# Autodesk Inventor assembly: これで完成パネル型スカラアーム
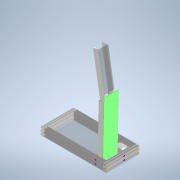
[picture p0: Inventor's stored thumbnail of the model, 180x180]
Saved by Autodesk Inventor 2022 (Build 260153000, 153)
## iProperties
Created: 2022-12-16
Part Number: これで完成パネル型スカラアーム
Document SubType Name: Assembly
Designer: tdn82
Author: tdn82
## Documents named in this file (21)
- C:\Users\tdn82\OneDrive\ドキュメント\Inventor\卒業研究パネル型スカラアーム\GrabCAD\panel-type-scalar-arm\パネル型スカラアーム\サーボ固定パーツ３Dプリンタ出力実験\これで完成パネル型スカラアーム.iam
- C:\Users\tdn82\OneDrive\ドキュメント\Inventor\卒業研究パネル型スカラアーム\GrabCAD\panel-type-scalar-arm\パネル型スカラアーム\後ろカバー.ipt
- C:\Users\tdn82\OneDrive\ドキュメント\Inventor\卒業研究パネル型スカラアーム\GrabCAD\panel-type-scalar-arm\パネル型スカラアーム\HFS5-2040-180-Z5-YA10-YB99-YC170.ipt
- C:\Users\tdn82\OneDrive\ドキュメント\Inventor\卒業研究パネル型スカラアーム\GrabCAD\panel-type-scalar-arm\パネル型スカラアーム\HFS5-2040-320-TPW-Z5-YA42_5.ipt
- C:\Users\tdn82\OneDrive\ドキュメント\Inventor\卒業研究パネル型スカラアーム\GrabCAD\panel-type-scalar-arm\パネル型スカラアーム\HFS5-2040-320-TPW.ipt
- C:\Users\tdn82\OneDrive\ドキュメント\Inventor\卒業研究パネル型スカラアーム\GrabCAD\panel-type-scalar-arm\パネル型スカラアーム\HFS5-2040-180-Z5-YA10-YB170-Left.ipt
- C:\Users\tdn82\OneDrive\ドキュメント\Inventor\卒業研究パネル型スカラアーム\GrabCAD\panel-type-scalar-arm\パネル型スカラアーム\サーボ固定パーツ３Dプリンタ出力実験\サーボモータ固定用１軸目.ipt
- C:\Users\tdn82\OneDrive\ドキュメント\Inventor\卒業研究パネル型スカラアーム\GrabCAD\panel-type-scalar-arm\パネル型スカラアーム\サーボモータB3M1000_scale.ipt
- C:\Users\tdn82\OneDrive\ドキュメント\Inventor\卒業研究パネル型スカラアーム\GrabCAD\panel-type-scalar-arm\パネル型スカラアーム\サーボ固定パーツ３Dプリンタ出力実験\シャフト固定用.ipt
- C:\Users\tdn82\OneDrive\ドキュメント\Inventor\卒業研究パネル型スカラアーム\GrabCAD\panel-type-scalar-arm\パネル型スカラアーム\横長2ndフラットバー上 アルミフレーム用.ipt
- C:\Users\tdn82\OneDrive\ドキュメント\Inventor\卒業研究パネル型スカラアーム\GrabCAD\panel-type-scalar-arm\パネル型スカラアーム\横長2ndフラットバー下 アルミフレーム用.ipt
- C:\Users\tdn82\OneDrive\ドキュメント\Inventor\卒業研究パネル型スカラアーム\GrabCAD\panel-type-scalar-arm\パネル型スカラアーム\前カバー中盤左アーム固定.ipt
- C:\Users\tdn82\OneDrive\ドキュメント\Inventor\卒業研究パネル型スカラアーム\GrabCAD\panel-type-scalar-arm\パネル型スカラアーム\サーボ固定パーツ３Dプリンタ出力実験\サーボモータ固定用２軸目3mm改_new.ipt
- C:\Users\tdn82\OneDrive\ドキュメント\Inventor\卒業研究パネル型スカラアーム\GrabCAD\panel-type-scalar-arm\パネル型スカラアーム\アルミフリーホーン02137_AluminumFreeHornWithBearing_B3M_6000.ipt
- C:\Users\tdn82\OneDrive\ドキュメント\Inventor\卒業研究パネル型スカラアーム\GrabCAD\panel-type-scalar-arm\パネル型スカラアーム\シャフト.ipt
- C:\Users\tdn82\OneDrive\ドキュメント\Inventor\卒業研究パネル型スカラアーム\GrabCAD\panel-type-scalar-arm\パネル型スカラアーム\FL674ZZ.ipt
- C:\Users\tdn82\OneDrive\ドキュメント\Inventor\卒業研究パネル型スカラアーム\GrabCAD\panel-type-scalar-arm\パネル型スカラアーム\シャフトカラー.ipt
- C:\Users\tdn82\OneDrive\ドキュメント\Inventor\卒業研究パネル型スカラアーム\GrabCAD\panel-type-scalar-arm\パネル型スカラアーム\横長3rdフラットバー下.ipt
- C:\Users\tdn82\OneDrive\ドキュメント\Inventor\卒業研究パネル型スカラアーム\GrabCAD\panel-type-scalar-arm\パネル型スカラアーム\三段目アクリル板.ipt
- C:\Users\tdn82\OneDrive\ドキュメント\Inventor\卒業研究パネル型スカラアーム\GrabCAD\panel-type-scalar-arm\パネル型スカラアーム\CBE5-25.ipt
- C:\Users\tdn82\OneDrive\ドキュメント\Inventor\卒業研究パネル型スカラアーム\GrabCAD\panel-type-scalar-arm\パネル型スカラアーム\CBE5-20.ipt
## Components (32 placed, 20 different names)
1. 後ろカバー:3 — メイト:1, メイト:2, フラッシュ:1, メイト:3, フラッシュ:2, フラッシュ:4, メイト:17
2. HFS5-2040-180-Z5-YA10-YB99-YC170:1 — メイト:3, フラッシュ:2, メイト:6, フラッシュ:4, メイト:9, フラッシュ:6, メイト:11, 挿入:26, 挿入:27, 挿入:28, 挿入:29, 挿入:30, 挿入:31, フラッシュ:9, メイト:18, フラッシュ:10
3. HFS5-2040-320-TPW-Z5-YA42_5:1 — フラッシュ:9, メイト:18, フラッシュ:10, 挿入:32, 挿入:33, メイト:19, メイト:22
4. HFS5-2040-320-TPW:1 — メイト:2, フラッシュ:1, メイト:6, メイト:16, フラッシュ:8
5. HFS5-2040-180-Z5-YA10-YB170-Left:1 — メイト:16, メイト:17, フラッシュ:8, 挿入:22, 挿入:23, 挿入:24, 挿入:25
6. サーボモータ固定用１軸目:1 — メイト:9, フラッシュ:6, メイト:10, 挿入:1, 挿入:2, メイト:11
7. サーボモータB3M1000_scale:1 — メイト:10, 挿入:1, 挿入:2, 挿入:12
8. サーボモータB3M1000_scale:2 — 挿入:9, 挿入:10, 挿入:18, 挿入:19, 挿入:20
9. シャフト固定用:1 — メイト:19, メイト:20, メイト:21
10. 横長2ndフラットバー上 アルミフレーム用:1 — 挿入:3, 挿入:4, 挿入:12
11. 横長2ndフラットバー下 アルミフレーム用:1 — 挿入:13, 挿入:14, 挿入:15
12. 前カバー中盤左アーム固定:1 — 挿入:3, 挿入:4, 挿入:7, 挿入:8, 挿入:13, 挿入:14
13. サーボモータ固定用２軸目3mm改_new:1 — 挿入:7, 挿入:8, 挿入:9, 挿入:10
14. アルミフリーホーン02137_AluminumFreeHornWithBearing_B3M_6000:1 — 挿入:18
15. シャフト:1 — メイト:13, メイト:22
16. FL674ZZ:1 — 挿入:15, メイト:13, 挿入:17
17. シャフトカラー:1 — 挿入:17
18. 横長3rdフラットバー下:1 — 挿入:19, メイト:15
19. 横長3rdフラットバー下:2 — 挿入:20, メイト:14, フラッシュ:7, 挿入:21
20. 三段目アクリル板:1 — メイト:14, メイト:15, フラッシュ:7, 挿入:21
21. CBE5-25:1 — 挿入:23
22. CBE5-25:2 — 挿入:22
23. CBE5-25:3 — 挿入:25
24. CBE5-25:4 — 挿入:24
25. CBE5-25:5 — 挿入:26
26. CBE5-25:6 — 挿入:27
27. CBE5-25:7 — 挿入:28
28. CBE5-25:8 — 挿入:29
29. CBE5-20:1 — 挿入:30
30. CBE5-20:2 — 挿入:31
31. CBE5-20:3 — 挿入:33, メイト:21
32. CBE5-20:4 — 挿入:32, メイト:20
## Relationships (54: Insert 29, Mate 17, Flush 8)
- メイト:1 [Mate]: 後ろカバー:3
- メイト:2 [Mate]: 後ろカバー:3 ↔ HFS5-2040-320-TPW:1
- フラッシュ:1 [Flush]: 後ろカバー:3 ↔ HFS5-2040-320-TPW:1
- メイト:3 [Mate]: 後ろカバー:3 ↔ HFS5-2040-180-Z5-YA10-YB99-YC170:1
- フラッシュ:2 [Flush]: 後ろカバー:3 ↔ HFS5-2040-180-Z5-YA10-YB99-YC170:1
- メイト:6 [Mate]: HFS5-2040-180-Z5-YA10-YB99-YC170:1 ↔ HFS5-2040-320-TPW:1
- フラッシュ:4 [Flush]: 後ろカバー:3 ↔ HFS5-2040-180-Z5-YA10-YB99-YC170:1
- メイト:9 [Mate]: HFS5-2040-180-Z5-YA10-YB99-YC170:1 ↔ サーボモータ固定用１軸目:1
- フラッシュ:6 [Flush]: HFS5-2040-180-Z5-YA10-YB99-YC170:1 ↔ サーボモータ固定用１軸目:1
- メイト:10 [Mate]: サーボモータ固定用１軸目:1 ↔ サーボモータB3M1000_scale:1
- 挿入:1 [Insert]: サーボモータ固定用１軸目:1 ↔ サーボモータB3M1000_scale:1
- 挿入:2 [Insert]: サーボモータ固定用１軸目:1 ↔ サーボモータB3M1000_scale:1
- メイト:11 [Mate]: HFS5-2040-180-Z5-YA10-YB99-YC170:1 ↔ サーボモータ固定用１軸目:1
- 挿入:3 [Insert]: 横長2ndフラットバー上 アルミフレーム用:1 ↔ 前カバー中盤左アーム固定:1
- 挿入:4 [Insert]: 横長2ndフラットバー上 アルミフレーム用:1 ↔ 前カバー中盤左アーム固定:1
- 挿入:7 [Insert]: 前カバー中盤左アーム固定:1 ↔ サーボモータ固定用２軸目3mm改_new:1
- 挿入:8 [Insert]: 前カバー中盤左アーム固定:1 ↔ サーボモータ固定用２軸目3mm改_new:1
- 挿入:9 [Insert]: サーボモータB3M1000_scale:2 ↔ サーボモータ固定用２軸目3mm改_new:1
- 挿入:10 [Insert]: サーボモータB3M1000_scale:2 ↔ サーボモータ固定用２軸目3mm改_new:1
- 挿入:12 [Insert]: サーボモータB3M1000_scale:1 ↔ 横長2ndフラットバー上 アルミフレーム用:1
- 挿入:13 [Insert]: 横長2ndフラットバー下 アルミフレーム用:1 ↔ 前カバー中盤左アーム固定:1
- 挿入:14 [Insert]: 横長2ndフラットバー下 アルミフレーム用:1 ↔ 前カバー中盤左アーム固定:1
- 挿入:15 [Insert]: 横長2ndフラットバー下 アルミフレーム用:1 ↔ FL674ZZ:1
- メイト:13 [Mate]: シャフト:1 ↔ FL674ZZ:1
- 挿入:17 [Insert]: FL674ZZ:1 ↔ シャフトカラー:1
- 挿入:18 [Insert] (-1 mm): サーボモータB3M1000_scale:2 ↔ アルミフリーホーン02137_AluminumFreeHornWithBearing_B3M_6000:1
- 挿入:19 [Insert]: サーボモータB3M1000_scale:2 ↔ 横長3rdフラットバー下:1
- 挿入:20 [Insert] (-1 mm): サーボモータB3M1000_scale:2 ↔ 横長3rdフラットバー下:2
- メイト:14 [Mate]: 横長3rdフラットバー下:2 ↔ 三段目アクリル板:1
- メイト:15 [Mate]: 横長3rdフラットバー下:1 ↔ 三段目アクリル板:1
- フラッシュ:7 [Flush]: 横長3rdフラットバー下:2 ↔ 三段目アクリル板:1
- 挿入:21 [Insert]: 横長3rdフラットバー下:2 ↔ 三段目アクリル板:1
- メイト:16 [Mate]: HFS5-2040-320-TPW:1 ↔ HFS5-2040-180-Z5-YA10-YB170-Left:1
- メイト:17 [Mate]: 後ろカバー:3 ↔ HFS5-2040-180-Z5-YA10-YB170-Left:1
- フラッシュ:8 [Flush]: HFS5-2040-320-TPW:1 ↔ HFS5-2040-180-Z5-YA10-YB170-Left:1
- 挿入:22 [Insert]: HFS5-2040-180-Z5-YA10-YB170-Left:1 ↔ CBE5-25:2
- 挿入:23 [Insert]: HFS5-2040-180-Z5-YA10-YB170-Left:1 ↔ CBE5-25:1
- 挿入:24 [Insert]: HFS5-2040-180-Z5-YA10-YB170-Left:1 ↔ CBE5-25:4
- 挿入:25 [Insert]: HFS5-2040-180-Z5-YA10-YB170-Left:1 ↔ CBE5-25:3
- 挿入:26 [Insert]: HFS5-2040-180-Z5-YA10-YB99-YC170:1 ↔ CBE5-25:5
- 挿入:27 [Insert]: HFS5-2040-180-Z5-YA10-YB99-YC170:1 ↔ CBE5-25:6
- 挿入:28 [Insert]: HFS5-2040-180-Z5-YA10-YB99-YC170:1 ↔ CBE5-25:7
- 挿入:29 [Insert]: HFS5-2040-180-Z5-YA10-YB99-YC170:1 ↔ CBE5-25:8
- 挿入:30 [Insert]: HFS5-2040-180-Z5-YA10-YB99-YC170:1 ↔ CBE5-20:1
- 挿入:31 [Insert]: HFS5-2040-180-Z5-YA10-YB99-YC170:1 ↔ CBE5-20:2
- フラッシュ:9 [Flush]: HFS5-2040-180-Z5-YA10-YB99-YC170:1 ↔ HFS5-2040-320-TPW-Z5-YA42_5:1
- メイト:18 [Mate]: HFS5-2040-180-Z5-YA10-YB99-YC170:1 ↔ HFS5-2040-320-TPW-Z5-YA42_5:1
- フラッシュ:10 [Flush]: HFS5-2040-180-Z5-YA10-YB99-YC170:1 ↔ HFS5-2040-320-TPW-Z5-YA42_5:1
- 挿入:32 [Insert]: HFS5-2040-320-TPW-Z5-YA42_5:1 ↔ CBE5-20:4
- 挿入:33 [Insert]: HFS5-2040-320-TPW-Z5-YA42_5:1 ↔ CBE5-20:3
- メイト:19 [Mate]: HFS5-2040-320-TPW-Z5-YA42_5:1 ↔ シャフト固定用:1
- メイト:20 [Mate]: シャフト固定用:1 ↔ CBE5-20:4
- メイト:21 [Mate]: シャフト固定用:1 ↔ CBE5-20:3
- メイト:22 [Mate]: HFS5-2040-320-TPW-Z5-YA42_5:1 ↔ シャフト:1
